# Autodesk Inventor assembly: FNAL Gantry Table With Chucks - V2F
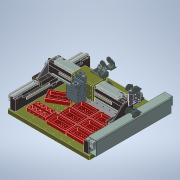
[picture p0: Inventor's stored thumbnail of the model, 180x180]
Saved by Autodesk Inventor 2022 (Build 260153000, 153)
## iProperties
Created: 2021-03-05
Part Number: FNAL Gantry Table With Chucks - V2F
Document SubType Name: Assembly
Designer: caleb
Author: caleb
## Documents named in this file (5)
- C:\Users\Caleb\Desktop\nebraska-silicon-lab\Hardware\ETL\Module Assembly\FNAL Gantry Table With Chucks - V2F.iam
- C:\Users\Caleb\Desktop\nebraska-silicon-lab\Hardware\ETL\FNAL Gantry\F10129268--_1-ASSY_ CMS2 ETL_ SMALLER AEROTECH GANTRY TOP LEVEL ASSEMBLY __ES13805-1__stp.iam
- C:\Users\Caleb\Desktop\nebraska-silicon-lab\Hardware\ETL\Module Assembly\Chuck - V2F\Chuck - V2F.iam
- C:\Users\Caleb\Desktop\nebraska-silicon-lab\Hardware\General Gantry\Gantry Tool Rack\Tool Rack Assembly.iam
- C:\Users\Caleb\Desktop\nebraska-silicon-lab\Hardware\ETL\Module Assembly\Chuck - OctopocketF\Chuck - OctopocketF.iam
## Components (10 placed, 4 different names)
1. F10129268--_1-ASSY_ CMS2 ETL_ SMALLER AEROTECH GANTRY TOP LEVEL ASSEMBLY __ES13805-1__stp:1 [sub-assembly] — Mate:1, Mate:2, Mate:3, Mate:5, Mate:6, Mate:7, Mate:8, Angle:2, Mate:10, Angle:3
2. Chuck - V2F:1 [sub-assembly] — Mate:2
3. Chuck - V2F:2 [sub-assembly] — Mate:3
4. Chuck - V2F:3 [sub-assembly] — Mate:1
5. Tool Rack Assembly:1 [sub-assembly] — Mate:10
6. Chuck - V2F:5 [sub-assembly] — Mate:7, Angle:2
7. Chuck - V2F:6 [sub-assembly] — Mate:8
8. Chuck - V2F:7 [sub-assembly] — Mate:5
9. Chuck - V2F:9 [sub-assembly] — Mate:6
10. Chuck - OctopocketF:1 [sub-assembly] — Angle:3
## Relationships (10: Mate 8, Angle 2)
- Mate:1: F10129268--_1-ASSY_ CMS2 ETL_ SMALLER AEROTECH GANTRY TOP LEVEL ASSEMBLY __ES13805-1__stp:1 ↔ Chuck - V2F:3
- Mate:2: F10129268--_1-ASSY_ CMS2 ETL_ SMALLER AEROTECH GANTRY TOP LEVEL ASSEMBLY __ES13805-1__stp:1 ↔ Chuck - V2F:1
- Mate:3: F10129268--_1-ASSY_ CMS2 ETL_ SMALLER AEROTECH GANTRY TOP LEVEL ASSEMBLY __ES13805-1__stp:1 ↔ Chuck - V2F:2
- Mate:5: F10129268--_1-ASSY_ CMS2 ETL_ SMALLER AEROTECH GANTRY TOP LEVEL ASSEMBLY __ES13805-1__stp:1 ↔ Chuck - V2F:7
- Mate:6: F10129268--_1-ASSY_ CMS2 ETL_ SMALLER AEROTECH GANTRY TOP LEVEL ASSEMBLY __ES13805-1__stp:1 ↔ Chuck - V2F:9
- Mate:7: F10129268--_1-ASSY_ CMS2 ETL_ SMALLER AEROTECH GANTRY TOP LEVEL ASSEMBLY __ES13805-1__stp:1 ↔ Chuck - V2F:5
- Mate:8: F10129268--_1-ASSY_ CMS2 ETL_ SMALLER AEROTECH GANTRY TOP LEVEL ASSEMBLY __ES13805-1__stp:1 ↔ Chuck - V2F:6
- Angle:2 (0 deg): F10129268--_1-ASSY_ CMS2 ETL_ SMALLER AEROTECH GANTRY TOP LEVEL ASSEMBLY __ES13805-1__stp:1 ↔ Chuck - V2F:5
- Mate:10: F10129268--_1-ASSY_ CMS2 ETL_ SMALLER AEROTECH GANTRY TOP LEVEL ASSEMBLY __ES13805-1__stp:1 ↔ Tool Rack Assembly:1
- Angle:3 (0 deg): F10129268--_1-ASSY_ CMS2 ETL_ SMALLER AEROTECH GANTRY TOP LEVEL ASSEMBLY __ES13805-1__stp:1 ↔ Chuck - OctopocketF:1
